# Autodesk Inventor assembly: LG_CRD_8521B
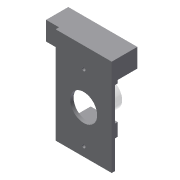
[picture p0: Inventor's stored thumbnail of the model, 180x180]
Saved by Autodesk Inventor 2019 (Build 230136000, 136)
## iProperties
Created: 2019-06-12
Part Number: LG_CRD_8521B
Document SubType Name: Assembly
Designer: diederichbenedict
Author: diederichbenedict
## Documents named in this file (3)
- C:\Users\diederichbenedict\Dropbox\Dokumente\Promotion\PROJECTS\STORMoChip\INVENTOR\Nanoscopy-on-a-cheap\LG_CRD_8521B.iam
- C:\Users\diederichbenedict\Dropbox\Dokumente\Promotion\PROJECTS\STORMoChip\INVENTOR\Nanoscopy-on-a-cheap\LG_CRD_8521B_Lens.ipt
- C:\Users\diederichbenedict\Dropbox\Dokumente\Promotion\PROJECTS\STORMoChip\INVENTOR\Nanoscopy-on-a-cheap\LG_CRD_8521B_Base.ipt
## Components (2 placed, 2 different names)
1. LG_CRD_8521B_Lens:1 — Mate:1, Flush:1
2. LG_CRD_8521B_Base:1 — Mate:1, Flush:1
## Relationships (2: Mate 1, Flush 1)
- Mate:1: LG_CRD_8521B_Lens:1 ↔ LG_CRD_8521B_Base:1
- Flush:1: LG_CRD_8521B_Lens:1 ↔ LG_CRD_8521B_Base:1
